# Autodesk Inventor assembly: AMR
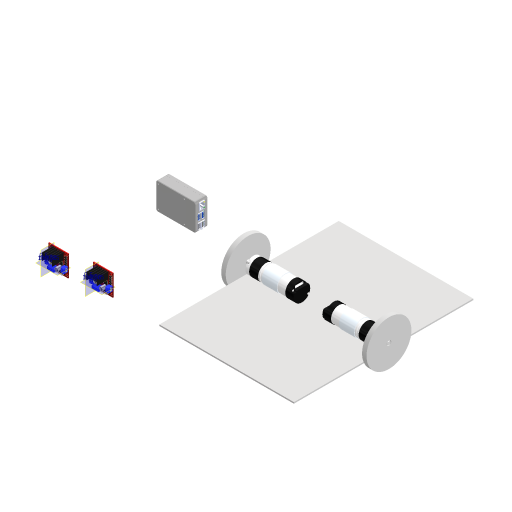
[picture p0: Inventor's stored thumbnail of the model, 512x512]
Saved by Autodesk Inventor 2024.2 (Build 282272000, 272)
## iProperties
Created: 2025-01-10
Part Number: AMR
Document SubType Name: Assembly
Designer: Kartik
Mass: 817.853 g
Surface Area: 4392.15 cm^2
Volume: 808.976 cm^3
Density: 1.01097 g/cm^3
Author: Kartik
## Documents named in this file (7)
- D:\Kartik\AMR\Basic_Robot\CAD\Assemblies\AMR.iam
- D:\Kartik\AMR\Basic_Robot\CAD\Boughtouts\Planetarygear_Motor.iam
- D:\Kartik\AMR\Basic_Robot\CAD\Parts\AMR_Base.ipt
- D:\Kartik\AMR\Basic_Robot\CAD\Parts\Wheel.ipt
- D:\Kartik\AMR\Basic_Robot\CAD\Boughtouts\h-bridge-L298n\H-brug.ipt
- D:\Kartik\AMR\Basic_Robot\CAD\Boughtouts\raspberry-pi-4-model-b\Raspberry Pi 4 Model B\Raspberry Pi 4 Model B.ipt
- D:\Kartik\AMR\Basic_Robot\CAD\Boughtouts\raspberry-pi-4-model-b-case\Raspberry_pi_4_case v2\Raspberry_pi_4_case v2.ipt
## Components (9 placed, 6 different names)
1. Planetarygear_Motor:1 [sub-assembly] — Mate:1, Flush:2, Mate:4, Angle:2, Mate:5, Angle:3
2. Planetarygear_Motor:2 [sub-assembly] — Mate:2, Flush:1, Mate:5, Mate:8, Angle:4
3. AMR_Base:1 — Mate:3, Angle:1, Angle:2, Mate:6, Mate:7, Mate:8, Angle:3, Angle:4
4. Wheel:1 — Mate:1, Flush:2, Mate:6
5. Wheel:2 — Mate:2, Flush:1, Mate:7
6. H-brug:1
7. H-brug:2
8. Raspberry Pi 4 Model B:1 — Mate:10, Mate:11
9. Raspberry_pi_4_case v2:1 — Mate:10, Mate:11
## Relationships (16: Mate 10, Angle 4, Flush 2)
- Mate:1: Planetarygear_Motor:1 ↔ Wheel:1
- Mate:2: Planetarygear_Motor:2 ↔ Wheel:2
- Flush:1: Planetarygear_Motor:2 ↔ Wheel:2
- Flush:2: Planetarygear_Motor:1 ↔ Wheel:1
- Mate:3: AMR_Base:1
- Angle:1 (0 deg): AMR_Base:1
- Mate:4: Planetarygear_Motor:1
- Angle:2 (-90 deg): Planetarygear_Motor:1 ↔ AMR_Base:1
- Mate:5: Planetarygear_Motor:1 ↔ Planetarygear_Motor:2
- Mate:6 (2 mm): AMR_Base:1 ↔ Wheel:1
- Mate:7 (2 mm): AMR_Base:1 ↔ Wheel:2
- Mate:8 (20 mm): Planetarygear_Motor:2 ↔ AMR_Base:1
- Angle:3 (0 deg): Planetarygear_Motor:1 ↔ AMR_Base:1
- Angle:4 (0 deg): Planetarygear_Motor:2 ↔ AMR_Base:1
- Mate:10: Raspberry Pi 4 Model B:1 ↔ Raspberry_pi_4_case v2:1
- Mate:11: Raspberry Pi 4 Model B:1 ↔ Raspberry_pi_4_case v2:1
